# Autodesk Inventor assembly: Case
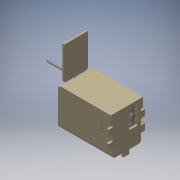
[picture p0: Inventor's stored thumbnail of the model, 180x180]
Saved by Autodesk Inventor 2019 (Build 230136000, 136)
## iProperties
Created: 2019-02-19
Part Number: Case
Material: 일반
Document SubType Name: Assembly
Designer: Jeong Ji Hoon
Author: Jeong Ji Hoon
## Documents named in this file (8)
- C:\VCF\Microdrive\Case.iam
- C:\VCF\Microdrive\Millmax.ipt
- C:\VCF\Microdrive\PCB.ipt
- C:\VCF\Microdrive\PCB_Holder.ipt
- C:\VCF\Microdrive\Assembly.iam
- C:\VCF\Microdrive\Case_Body.ipt
- C:\VCF\Microdrive\Case_Side.ipt
- C:\VCF\Microdrive\Case_Top.ipt
## Components (7 placed, 7 different names)
1. Assembly:1 [sub-assembly] — 강체:3
2. Millmax:1 — 강체:1
3. PCB:1 — 강체:1, 강체:5
4. PCB_Holder:1 — 강체:3, 강체:4, 강체:5
5. Case_Body:1 — 강체:4, 강체:6, 슬라이더:1
6. Case_Side:1 — 강체:6
7. Case_Top:1 — 슬라이더:1
## Relationships (6: WeldJoint 5, TranslationJoint 1)
- 강체:1 [WeldJoint]: Millmax:1 ↔ PCB:1
- 강체:3 [WeldJoint]: Assembly:1 ↔ PCB_Holder:1
- 강체:4 [WeldJoint]: PCB_Holder:1 ↔ Case_Body:1
- 강체:5 [WeldJoint]: PCB:1 ↔ PCB_Holder:1
- 강체:6 [WeldJoint]: Case_Body:1 ↔ Case_Side:1
- 슬라이더:1 [TranslationJoint] (0.25 mm): Case_Body:1 ↔ Case_Top:1
